# Autodesk Inventor assembly: Assembly1
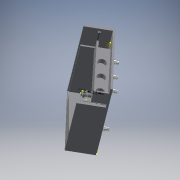
[picture p0: Inventor's stored thumbnail of the model, 180x180]
Saved by Autodesk Inventor 2019 (Build 230136000, 136)
## iProperties
Created: 2020-02-20
Part Number: Assembly1
Document SubType Name: Assembly
Designer: LENOVO
Author: LENOVO
## Documents named in this file (10)
- C:\Users\LENOVO\Desktop\Abhishek\Assembly1.iam
- C:\Users\LENOVO\Desktop\Abhishek\base part.ipt
- C:\Users\LENOVO\Desktop\Abhishek\dc motor.ipt
- C:\Users\LENOVO\Desktop\Abhishek\ball pickr.ipt
- C:\Users\LENOVO\Desktop\Abhishek\Bracket.ipt
- C:\Users\LENOVO\Desktop\Abhishek\14Screw92005A124.ipt
- C:\Users\LENOVO\Desktop\Abhishek\checking.ipt
- C:\Users\LENOVO\Desktop\Abhishek\comp convey.iam
- C:\Users\LENOVO\Desktop\Abhishek\roller shaft.ipt
- C:\Users\LENOVO\Desktop\Abhishek\closing.ipt
## Components (25 placed, 9 different names)
1. base part:1 — Mate:1, Mate:2, Mate:3, Mate:4, Mate:5, Mate:6, Mate:7, Mate:8, Mate:16, Mate:17, Mate:18, Mate:19, Mate:23, Mate:24, Mate:25, Mate:26, Mate:27, Mate:28, Mate:29, Mate:30, Mate:31, Mate:35, Mate:36, Mate:37, Mate:38, Mate:39, Mate:41, Mate:44, Mate:47, Mate:50, Mate:51, Mate:52, Mate:53, Mate:54, Mate:55, Mate:56, Mate:57, Mate:60, Mate:61
2. dc motor:1 — Mate:3, Mate:6, Mate:68, Mate:69
3. dc motor:2 — Mate:2, Mate:4, Mate:64, Mate:65
4. dc motor:3 — Mate:1, Mate:5, Mate:66, Mate:67
5. dc motor:4 — Mate:7, Mate:8, Mate:9, Mate:10
6. ball pickr:1 — Mate:9, Mate:10
7. Bracket:5 — Mate:16, Mate:17, Mate:42, Mate:43
8. Bracket:8 — Mate:29, Mate:39, Mate:53
9. Bracket:10 — Mate:19, Mate:36, Mate:44, Mate:45, Mate:46
10. Bracket:11 — Mate:25, Mate:26, Mate:51
11. Bracket:12 — Mate:31, Mate:38, Mate:54
12. Bracket:13 — Mate:30, Mate:35, Mate:55
13. Bracket:14 — Mate:18, Mate:37, Mate:47, Mate:48, Mate:49
14. Bracket:15 — Mate:27, Mate:28, Mate:50
15. Bracket:16 — Mate:23, Mate:24, Mate:52
16. 14Screw92005A124:1 — Mate:41, Mate:42, Mate:43
17. 14Screw92005A124:2 — Mate:45, Mate:46
18. 14Screw92005A124:3 — Mate:48, Mate:49
19. checking:1 — Mate:56, Mate:57, Mate:58, Mate:59
20. comp convey:1 [sub-assembly] — Mate:58, Mate:59, Mate:62, Mate:63
21. roller shaft:1 — Mate:62, Mate:63
22. dc motor:5 — Mate:60, Mate:61
23. closing:1 — Mate:64, Mate:65
24. closing:2 — Mate:66, Mate:67
25. closing:3 — Mate:68, Mate:69
## Relationships (57: Mate 57)
- Mate:1: base part:1 ↔ dc motor:3
- Mate:2: base part:1 ↔ dc motor:2
- Mate:3: base part:1 ↔ dc motor:1
- Mate:4: base part:1 ↔ dc motor:2
- Mate:5: base part:1 ↔ dc motor:3
- Mate:6: base part:1 ↔ dc motor:1
- Mate:7: base part:1 ↔ dc motor:4
- Mate:8: base part:1 ↔ dc motor:4
- Mate:9: dc motor:4 ↔ ball pickr:1
- Mate:10: dc motor:4 ↔ ball pickr:1
- Mate:16: base part:1 ↔ Bracket:5
- Mate:17: base part:1 ↔ Bracket:5
- Mate:18: base part:1 ↔ Bracket:14
- Mate:19: base part:1 ↔ Bracket:10
- Mate:23: base part:1 ↔ Bracket:16
- Mate:24: base part:1 ↔ Bracket:16
- Mate:25: base part:1 ↔ Bracket:11
- Mate:26: base part:1 ↔ Bracket:11
- Mate:27: base part:1 ↔ Bracket:15
- Mate:28: base part:1 ↔ Bracket:15
- Mate:29: base part:1 ↔ Bracket:8
- Mate:30: base part:1 ↔ Bracket:13
- Mate:31: base part:1 ↔ Bracket:12
- Mate:35: base part:1 ↔ Bracket:13
- Mate:36: base part:1 ↔ Bracket:10
- Mate:37: base part:1 ↔ Bracket:14
- Mate:38: base part:1 ↔ Bracket:12
- Mate:39: base part:1 ↔ Bracket:8
- Mate:41: base part:1 ↔ 14Screw92005A124:1
- Mate:42: Bracket:5 ↔ 14Screw92005A124:1
- Mate:43: Bracket:5 ↔ 14Screw92005A124:1
- Mate:44: base part:1 ↔ Bracket:10
- Mate:45: Bracket:10 ↔ 14Screw92005A124:2
- Mate:46: Bracket:10 ↔ 14Screw92005A124:2
- Mate:47: base part:1 ↔ Bracket:14
- Mate:48: Bracket:14 ↔ 14Screw92005A124:3
- Mate:49: Bracket:14 ↔ 14Screw92005A124:3
- Mate:50: base part:1 ↔ Bracket:15
- Mate:51: base part:1 ↔ Bracket:11
- Mate:52: base part:1 ↔ Bracket:16
- Mate:53: base part:1 ↔ Bracket:8
- Mate:54: base part:1 ↔ Bracket:12
- Mate:55: base part:1 ↔ Bracket:13
- Mate:56: base part:1 ↔ checking:1
- Mate:57: base part:1 ↔ checking:1
- Mate:58: checking:1 ↔ comp convey:1
- Mate:59: checking:1 ↔ comp convey:1
- Mate:60: base part:1 ↔ dc motor:5
- Mate:61: base part:1 ↔ dc motor:5
- Mate:62: comp convey:1 ↔ roller shaft:1
- Mate:63: comp convey:1 ↔ roller shaft:1
- Mate:64: dc motor:2 ↔ closing:1
- Mate:65: dc motor:2 ↔ closing:1
- Mate:66: dc motor:3 ↔ closing:2
- Mate:67: dc motor:3 ↔ closing:2
- Mate:68: dc motor:1 ↔ closing:3
- Mate:69: dc motor:1 ↔ closing:3
